# Autodesk Inventor assembly: Assembly_Cube_AlliedVision_Alvium_v3_2
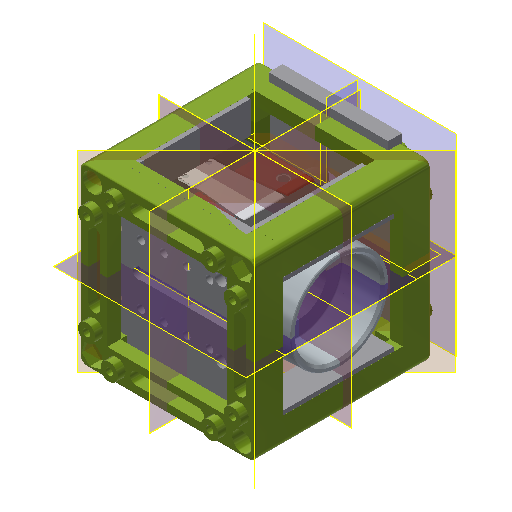
[picture p0: Inventor's stored thumbnail of the model, 512x512]
Saved by Autodesk Inventor 2023 (Build 270158000, 158)
## iProperties
Created: 2019-07-23
Part Number: Assembly_Cube_AlliedVision_Alvium_v3_2
Document SubType Name: Assembly
Designer: marsikovabarbora
Mass: 41.9543 g
Surface Area: 260.494 cm^2
Volume: 37.9382 cm^3
Density: 1.10586 g/cm^3
Author: marsikovabarbora
## Documents named in this file (6)
- C:\Users\diederichbenedict\Downloads\UC2 setup design\UC2 setup design\Assembly_Cube_AlliedVision_Alvium_v3.iam
- C:\Users\diederichbenedict\Downloads\UC2 setup design\UC2 setup design\20_Cube_insert_AlliedVision_Alvium_v3.ipt
- C:\Users\diederichbenedict\Downloads\UC2 setup design\UC2 setup design\Assembly_Cube_empty_IM_v3.iam
- C:\Users\diederichbenedict\Downloads\UC2 setup design\UC2 setup design\00_Basler_ace_USB3_C-Mount.ipt
- C:\Users\diederichbenedict\Downloads\UC2 setup design\UC2 setup design\20_Cube_Insert_Cmount_v3.ipt
- C:\Users\diederichbenedict\Downloads\UC2 setup design\UC2 setup design\00_Alvium_Step_USB90_S-Mount_ClosedHousing_2019-Mar-28.ipt
## Components (5 placed, 5 different names)
1. Assembly_Cube_empty_IM_v3:1 [sub-assembly] — Winkel:1, Winkel:2, Passend:1, Passend:2, Passend:3, Mate:4
2. 20_Cube_insert_AlliedVision_Alvium_v3:1 — Passend:1, Passend:2, Passend:3
3. 00_Basler_ace_USB3_C-Mount:1 — Winkel:1, Winkel:2
4. 20_Cube_Insert_Cmount_v3:1
5. 00_Alvium_Step_USB90_S-Mount_ClosedHousing_2019-Mar-28:1 — Mate:4
## Relationships (6: Mate 4, Angle 2)
- Winkel:1 [Angle] (0 deg): Assembly_Cube_empty_IM_v3:1 ↔ 00_Basler_ace_USB3_C-Mount:1
- Winkel:2 [Angle] (0 deg): Assembly_Cube_empty_IM_v3:1 ↔ 00_Basler_ace_USB3_C-Mount:1
- Passend:1 [Mate]: Assembly_Cube_empty_IM_v3:1 ↔ 20_Cube_insert_AlliedVision_Alvium_v3:1
- Passend:2 [Mate]: Assembly_Cube_empty_IM_v3:1 ↔ 20_Cube_insert_AlliedVision_Alvium_v3:1
- Passend:3 [Mate]: Assembly_Cube_empty_IM_v3:1 ↔ 20_Cube_insert_AlliedVision_Alvium_v3:1
- Mate:4: Assembly_Cube_empty_IM_v3:1 ↔ 00_Alvium_Step_USB90_S-Mount_ClosedHousing_2019-Mar-28:1
